# Autodesk Inventor assembly: Output
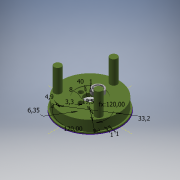
[picture p0: Inventor's stored thumbnail of the model, 180x180]
Saved by Autodesk Inventor 2018.3 (Build 223284000, 284)
## iProperties
Created: 2018-08-03
Part Number: Output
Material: Generisch
Document SubType Name: Assembly
Designer: JochenAlt
Author: JochenAlt
## Documents named in this file (4)
- D:\Projects\FlowerPot\CAD\CycloidalGear2\Output.iam
- D:\Projects\FlowerPot\CAD\CycloidalGear2\Output.ipt
- D:\Projects\FlowerPot\CAD\Mounting Hub.ipt
- C:\Users\JochenAlt\Documents\Inventor\Content Center Files\R2018\de-DE\SKF - Single row ball bearings\SKF60_2.5.ipt
## Components (3 placed, 3 different names)
1. Output:1 — Passend:1, Passend:2, Passend:3, Passend:4, Passend:5, Einfügen:1
2. Mounting Hub:1 — Passend:1, Passend:2, Passend:3, Passend:4, Passend:5
3. SKF- Kugellager, einreihig SKF60/2.5:1 — Einfügen:1
## Relationships (6: Mate 5, Insert 1)
- Passend:1 [Mate]: Output:1 ↔ Mounting Hub:1
- Passend:2 [Mate]: Output:1 ↔ Mounting Hub:1
- Passend:3 [Mate]: Output:1 ↔ Mounting Hub:1
- Passend:4 [Mate]: Output:1 ↔ Mounting Hub:1
- Passend:5 [Mate]: Output:1 ↔ Mounting Hub:1
- Einfügen:1 [Insert]: Output:1 ↔ SKF- Kugellager, einreihig SKF60/2.5:1
